# Autodesk Inventor assembly: Lower Platform
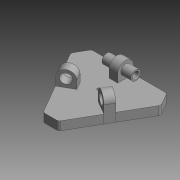
[picture p0: Inventor's stored thumbnail of the model, 180x180]
Saved by Autodesk Inventor 2014 SP1 (Build 180222100, 222)
## iProperties
Created: 2013-12-29
Part Number: Lower Platform
Document SubType Name: Assembly
Designer: tom
Author: tom
## Documents named in this file (4)
- C:\Users\tom\Documents\GitHub\Delta_Robots\Delatabot - Small Model\Inventor\Deltabot - Small Model\Lower Platform.iam
- C:\Users\tom\Documents\GitHub\Delta_Robots\Delatabot - Small Model\Inventor\Deltabot - Small Model\Lower Platform.ipt
- C:\Users\tom\Documents\GitHub\Delta_Robots\Delatabot - Small Model\Inventor\Deltabot - Small Model\Lower Arm Bracket.ipt
- C:\Users\tom\Documents\GitHub\Delta_Robots\Delatabot - Small Model\Inventor\Deltabot - Small Model\Linkage Mount.ipt
## Components (7 placed, 3 different names)
1. Lower Base
2. Lower Arm Bracket:1 — Mate:4, Mate:5
3. Lower Arm Bracket:2
4. Lower Arm Bracket:3
5. Linkage Mount:1 — Mate:4, Mate:5
6. Linkage Mount:2
7. Linkage Mount:3
## Component patterns: (3 elements, first: Lower Arm Bracket:1), (3 elements, first: Linkage Mount:1)
## Relationships (5: Mate 5)
- [Mate]: Lower Base ↔ Lower Arm Bracket:1
- [Mate]: Lower Base ↔ Lower Arm Bracket:1
- [Mate]: Lower Base ↔ Lower Arm Bracket:1
- Mate:4: Lower Arm Bracket:1 ↔ Linkage Mount:1
- Mate:5 (6.67 mm): Lower Arm Bracket:1 ↔ Linkage Mount:1
